# Autodesk Inventor assembly: downLow
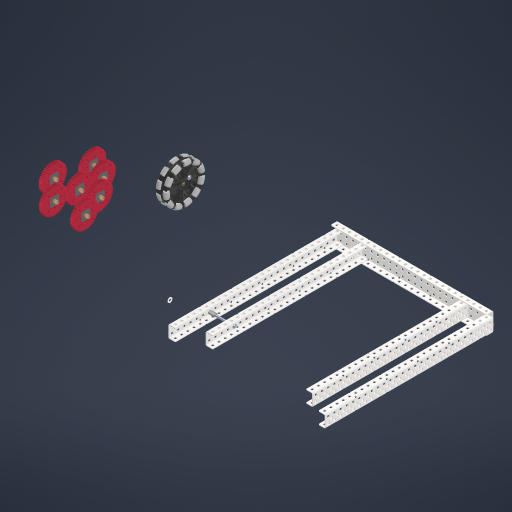
[picture p0: Inventor's stored thumbnail of the model, 512x512]
Saved by Autodesk Inventor 2023.4 (Build 274418000, 418)
## iProperties
Created: 2024-03-08
Part Number: downLow
Document SubType Name: Assembly
Designer: Meer
Author: Meer
## Documents named in this file (16)
- C:\Users\Meer\OneDrive\Documents\worlds bot possibly\downLow.iam
- C:\Users\Meer\OneDrive\Documents\GitHub\2024-599Z\Cad\Library\VEX-CAD-Inventor-1.4.0\Structure\C Channel\Aluminum 1x3x1\Alu C 1x3x1x25.ipt
- C:\Users\Meer\OneDrive\Documents\GitHub\2024-599Z\Cad\Library\VEX-CAD-Inventor-1.4.0\Structure\C Channel\Aluminum 1x2x1\Alu C 1x2x1x25.ipt
- C:\Users\Meer\OneDrive\Documents\GitHub\2024-599Z\Cad\Library\VEX-CAD-Inventor-1.4.0\Structure\C Channel\Aluminum 1x2x1\Alu C 1x2x1x27.ipt
- C:\Users\Meer\OneDrive\Documents\GitHub\2024-599Z\Cad\Library\VEX-CAD-Inventor-1.4.0\Structure\Hardware\Screw Steel - Star.ipt
- C:\Users\Meer\OneDrive\Documents\GitHub\2024-599Z\Cad\Library\VEX-CAD-Inventor-1.4.0\Structure\Hardware\Nut Keps.ipt
- C:\Users\Meer\OneDrive\Documents\GitHub\2024-599Z\Cad\Library\VEX-CAD-Inventor-1.4.0\Structure\Standoff\Standoff .50.ipt
- C:\Users\Meer\OneDrive\Documents\GitHub\2024-599Z\Cad\Library\VEX-CAD-Inventor-1.4.0\Structure\Standoff.ipt
- C:\Users\Meer\OneDrive\Documents\GitHub\2024-599Z\Cad\Library\VEX-CAD-Inventor-1.4.0\Structure\Hardware\Screw Steel - Star\SScrew Star Smooth 1.750.ipt
- C:\Users\Meer\OneDrive\Documents\GitHub\2024-599Z\Cad\Library\VEX-CAD-Inventor-1.4.0\Structure\Hardware\Screw Steel - Star\SScrew Star Smooth .290.ipt
- C:\Users\Meer\OneDrive\Documents\GitHub\2024-599Z\Cad\Library\VEX-CAD-Inventor-1.4.0\Motion\Wheels\Omni Wheel\3.25 Omni AS, No Insert.iam
- C:\Users\Meer\OneDrive\Documents\GitHub\2024-599Z\Cad\Library\VEX-CAD-Inventor-1.4.0\Motion\Wheels\Omni Wheel.iam
- C:\Users\Meer\OneDrive\Documents\GitHub\2024-599Z\Cad\Library\VEX-CAD-Inventor-1.4.0\Motion\Spacers\Washer Teflon.ipt
- C:\Users\Meer\OneDrive\Documents\GitHub\2024-599Z\Cad\Library\VEX-CAD-Inventor-1.4.0\Motion\Spacers\Washer Teflon\TWasher .375 OD x .03125.ipt
- C:\Users\Meer\OneDrive\Documents\GitHub\2024-599Z\Cad\Library\VEX-CAD-Inventor-1.4.0\Structure\Hardware\Screw Steel - Star\SScrew Star Smooth 1.250.ipt
- C:\Users\Meer\OneDrive\Documents\worlds bot possibly\42tHalfcut.iam
## Components (20 placed, 11 different names)
1. Alu C 1x3x1x25:1 — Insert:3, Insert:4, Insert:7, Insert:8
2. Alu C 1x2x1x25:1 — Insert:3, Insert:6, Insert:11
3. Alu C 1x2x1x25:2 — Insert:4
4. Nut Keps:1 — Insert:6, Insert:17
5. Alu C 1x2x1x27:3 — Insert:8
6. Alu C 1x2x1x27:4 — Insert:7, Insert:10, Insert:12
7. Standoff .50:1 — Insert:10
8. SScrew Star Smooth 1.750:1 — Insert:11
9. SScrew Star Smooth .290:2 — Insert:12
10. TWasher .375 OD x .03125:2 — Insert:17
11. TWasher .375 OD x .03125:3
12. 3.25 Omni AS, No Insert:1 [sub-assembly] — Insert:20
13. SScrew Star Smooth 1.250:5 — Insert:20
14. 42tHalfcut:1 [sub-assembly]
15. 42tHalfcut:2 [sub-assembly]
16. 42tHalfcut:3 [sub-assembly]
17. 42tHalfcut:4 [sub-assembly]
18. 42tHalfcut:5 [sub-assembly]
19. 42tHalfcut:6 [sub-assembly]
20. 42tHalfcut:7 [sub-assembly]
## Relationships (10: Insert 10)
- Insert:3: Alu C 1x3x1x25:1 ↔ Alu C 1x2x1x25:1
- Insert:4: Alu C 1x3x1x25:1 ↔ Alu C 1x2x1x25:2
- Insert:6: Alu C 1x2x1x25:1 ↔ Nut Keps:1
- Insert:7: Alu C 1x3x1x25:1 ↔ Alu C 1x2x1x27:4
- Insert:8: Alu C 1x3x1x25:1 ↔ Alu C 1x2x1x27:3
- Insert:10: Alu C 1x2x1x27:4 ↔ Standoff .50:1
- Insert:11: Alu C 1x2x1x25:1 ↔ SScrew Star Smooth 1.750:1
- Insert:12: Alu C 1x2x1x27:4 ↔ SScrew Star Smooth .290:2
- Insert:17: Nut Keps:1 ↔ TWasher .375 OD x .03125:2
- Insert:20: 3.25 Omni AS, No Insert:1 ↔ SScrew Star Smooth 1.250:5
